# Autodesk Inventor assembly: spur_gear_m0.8-18.4
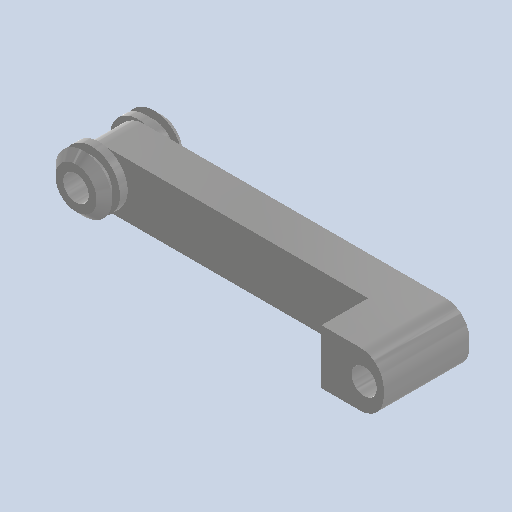
[picture p0: Inventor's stored thumbnail of the model, 512x512]
Saved by Autodesk Inventor 2025 (Build 290162000, 162)
## iProperties
Created: 2025-09-11
Part Number: spur_gear_m0.8-18.4
Document SubType Name: Assembly
Designer: sooo1
Author: sooo1
## Documents named in this file (3)
- C:\Users\sooo1\Documents\Inventor\MOBITOUCH\final\stroke_module_1\link_arm_b.iam
- C:\Users\sooo1\Documents\Inventor\MOBITOUCH\final\stroke_module_1\link_arm_b_1.ipt
- C:\Users\sooo1\Documents\Inventor\MOBITOUCH\final\stroke_module_1\spacer_Φ3.2_4.ipt
## Components (3 placed, 2 different names)
1. link_arm_b_1:1 — フラッシュ:1, フラッシュ:3, フラッシュ:4, フラッシュ:5, メイト:2, メイト:3, メイト:4
2. spacer_Φ3.2_4:1 — メイト:2, メイト:3
3. spacer_Φ3.2_4:2 — メイト:4
## Relationships (7: Flush 4, Mate 3)
- フラッシュ:1 [Flush]: link_arm_b_1:1
- フラッシュ:3 [Flush]: link_arm_b_1:1
- フラッシュ:4 [Flush]: link_arm_b_1:1
- フラッシュ:5 [Flush]: link_arm_b_1:1
- メイト:2 [Mate]: link_arm_b_1:1 ↔ spacer_Φ3.2_4:1
- メイト:3 [Mate]: link_arm_b_1:1 ↔ spacer_Φ3.2_4:1
- メイト:4 [Mate]: link_arm_b_1:1 ↔ spacer_Φ3.2_4:2
